# Autodesk Inventor assembly: TableGears
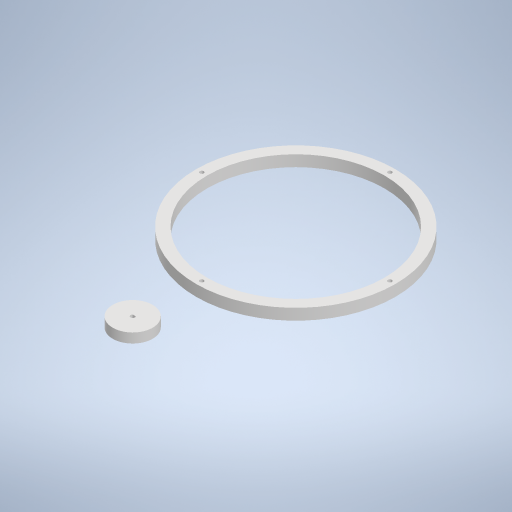
[picture p0: Inventor's stored thumbnail of the model, 512x512]
Saved by Autodesk Inventor 2023 (Build 270158000, 158)
## iProperties
Created: 2023-04-03
Part Number: TableGears
Document SubType Name: Assembly
Designer: czapa
Author: czapa
## Documents named in this file (3)
- C:\Users\czapa\OneDrive\Documents\GitHub\S.P.I.C.E\3D Models\Version1\TableGears.iam
- C:\Users\czapa\OneDrive\Documents\GitHub\S.P.I.C.E\3D Models\Version1\BearingTableGear.ipt
- C:\Users\czapa\OneDrive\Documents\GitHub\S.P.I.C.E\3D Models\Version1\motor_gearMK2.ipt
## Components (2 placed, 2 different names)
1. BearingTableGear:1 — Tangent:1, Flush:1
2. motor_gearMK2:1 — Tangent:1, Flush:1
## Relationships (2: Tangent 1, Flush 1)
- Tangent:1 (50 mm): BearingTableGear:1 ↔ motor_gearMK2:1
- Flush:1: BearingTableGear:1 ↔ motor_gearMK2:1
